# Autodesk Inventor assembly: Metal Scoop
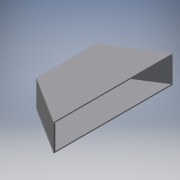
[picture p0: Inventor's stored thumbnail of the model, 180x180]
Saved by Autodesk Inventor 2017 (Build 210142000, 142)
## iProperties
Created: 2017-06-10
Part Number: Metal Scoop
Document SubType Name: Assembly
Designer: Matthew
Author: Matthew
## Documents named in this file (4)
- C:\Inventor Stuff\Robotics Trash\Metal Scoop\Metal Scoop.iam
- C:\Inventor Stuff\Robotics Trash\Metal Scoop\Top + Bottom.ipt
- C:\Inventor Stuff\Robotics Trash\Metal Scoop\Back Wall.ipt
- C:\Inventor Stuff\Robotics Trash\Metal Scoop\Side Wall.ipt
## Components (5 placed, 3 different names)
1. Top + Bottom:1 — Mate:1, Flush:1, Mate:2, Flush:2, Mate:3, Mate:4, Mate:5, Flush:3, Mate:6
2. Back Wall:1 — Mate:2, Flush:2, Mate:3, Flush:4
3. Side Wall:1 — Mate:1, Flush:1, Mate:4
4. Side Wall:2 — Mate:5, Flush:3, Mate:6, Mate:7, Flush:5
5. Top + Bottom:2 — Mate:7, Flush:4, Flush:5
## Relationships (12: Mate 7, Flush 5)
- Mate:1: Top + Bottom:1 ↔ Side Wall:1
- Flush:1: Top + Bottom:1 ↔ Side Wall:1
- Mate:2: Top + Bottom:1 ↔ Back Wall:1
- Flush:2: Top + Bottom:1 ↔ Back Wall:1
- Mate:3: Top + Bottom:1 ↔ Back Wall:1
- Mate:4: Top + Bottom:1 ↔ Side Wall:1
- Mate:5: Top + Bottom:1 ↔ Side Wall:2
- Flush:3: Top + Bottom:1 ↔ Side Wall:2
- Mate:6: Top + Bottom:1 ↔ Side Wall:2
- Mate:7: Side Wall:2 ↔ Top + Bottom:2
- Flush:4: Back Wall:1 ↔ Top + Bottom:2
- Flush:5: Side Wall:2 ↔ Top + Bottom:2
